# Autodesk Inventor assembly: Idler Front-Unit [B]
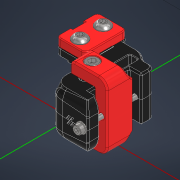
[picture p0: Inventor's stored thumbnail of the model, 180x180]
Saved by Autodesk Inventor 2022.2 (Build 262287010, 287A)
## iProperties
Created: 2022-03-14
Part Number: Idler Front-Unit [B]
Document SubType Name: Assembly
Designer: sleib
Author: sleib
## Documents named in this file (10)
- C:\Users\sleib\Projekte\Voron-2\CAD\Inventor\Idler Front-Unit [B].iam
- C:\Users\sleib\Projekte\Voron-2\CAD\Inventor\Idler Front Top [B].ipt
- C:\Users\sleib\Projekte\Voron-2\CAD\Inventor\Idler Front Bottom [B].ipt
- C:\Users\sleib\Projekte\Voron-2\CAD\Inventor\Idler Front Tensioner-Unit [B].iam
- C:\Users\sleib\Projekte\Voron-2\CAD\Inventor\M3x40 SHCS.ipt
- C:\Users\sleib\Projekte\Voron-2\CAD\Inventor\M5 Spacer (1mm).ipt
- C:\Users\sleib\Projekte\Voron-2\CAD\Inventor\Bearing F695-ZZ.ipt
- C:\Users\sleib\Projekte\Voron-2\CAD\Inventor\Z Belt-Clamp Upper.ipt
- C:\Users\sleib\Projekte\Voron-2\CAD\Inventor\M5x16 BHCS.ipt
- C:\Users\sleib\Projekte\Voron-2\CAD\Inventor\M3 Washer.ipt
## Components (12 placed, 9 different names)
1. Idler Front Top [B]:1 — Passend:1, Passend:3, Passend:5, Passend:6, Fluchtend:1, Winkel:1, Passend:8, Passend:11, Passend:19, Passend:22, Passend:25, Passend:26
2. Idler Front Bottom [B]:1 — Passend:5, Passend:6, Fluchtend:1, Passend:30, Passend:32
3. Idler Front Tensioner-Unit [B]:1 [sub-assembly] — Winkel:1, Passend:9, Passend:11, Passend:12, Passend:13, Passend:14, Passend:15
4. M3x40 SHCS:1 — Passend:8, Passend:9, Passend:29, Passend:31
5. M5 Spacer (1mm):1 — Passend:12, Passend:18, Passend:19
6. M5 Spacer (1mm):2 — Passend:15, Passend:16
7. Bearing F695-ZZ:1 — Passend:13, Passend:17, Passend:18
8. Bearing F695-ZZ:2 — Passend:14, Passend:16, Passend:17
9. Z Belt-Clamp Upper:1 — Passend:22, Passend:23, Passend:24, Passend:27, Passend:28
10. M5x16 BHCS:1 — Passend:23, Passend:25, Passend:27
11. M5x16 BHCS:2 — Passend:24, Passend:26, Passend:28
12. M3 Washer:1 — Passend:29, Passend:30, Passend:31
## Relationships (28: Mate 26, Flush 1, Angle 1)
- Passend:1 [Mate]: Idler Front Top [B]:1
- Passend:3 [Mate]: Idler Front Top [B]:1
- Passend:5 [Mate]: Idler Front Top [B]:1 ↔ Idler Front Bottom [B]:1
- Passend:6 [Mate]: Idler Front Top [B]:1 ↔ Idler Front Bottom [B]:1
- Fluchtend:1 [Flush]: Idler Front Top [B]:1 ↔ Idler Front Bottom [B]:1
- Winkel:1 [Angle] (0 deg): Idler Front Top [B]:1 ↔ Idler Front Tensioner-Unit [B]:1
- Passend:8 [Mate]: Idler Front Top [B]:1 ↔ M3x40 SHCS:1
- Passend:9 [Mate]: Idler Front Tensioner-Unit [B]:1 ↔ M3x40 SHCS:1
- Passend:11 [Mate] (5 mm): Idler Front Top [B]:1 ↔ Idler Front Tensioner-Unit [B]:1
- Passend:12 [Mate]: Idler Front Tensioner-Unit [B]:1 ↔ M5 Spacer (1mm):1
- Passend:13 [Mate]: Idler Front Tensioner-Unit [B]:1 ↔ Bearing F695-ZZ:1
- Passend:14 [Mate]: Idler Front Tensioner-Unit [B]:1 ↔ Bearing F695-ZZ:2
- Passend:15 [Mate]: Idler Front Tensioner-Unit [B]:1 ↔ M5 Spacer (1mm):2
- Passend:16 [Mate]: M5 Spacer (1mm):2 ↔ Bearing F695-ZZ:2
- Passend:17 [Mate]: Bearing F695-ZZ:1 ↔ Bearing F695-ZZ:2
- Passend:18 [Mate]: M5 Spacer (1mm):1 ↔ Bearing F695-ZZ:1
- Passend:19 [Mate]: Idler Front Top [B]:1 ↔ M5 Spacer (1mm):1
- Passend:22 [Mate]: Idler Front Top [B]:1 ↔ Z Belt-Clamp Upper:1
- Passend:23 [Mate]: Z Belt-Clamp Upper:1 ↔ M5x16 BHCS:1
- Passend:24 [Mate]: Z Belt-Clamp Upper:1 ↔ M5x16 BHCS:2
- Passend:25 [Mate]: Idler Front Top [B]:1 ↔ M5x16 BHCS:1
- Passend:26 [Mate]: Idler Front Top [B]:1 ↔ M5x16 BHCS:2
- Passend:27 [Mate]: Z Belt-Clamp Upper:1 ↔ M5x16 BHCS:1
- Passend:28 [Mate]: Z Belt-Clamp Upper:1 ↔ M5x16 BHCS:2
- Passend:29 [Mate]: M3x40 SHCS:1 ↔ M3 Washer:1
- Passend:30 [Mate]: Idler Front Bottom [B]:1 ↔ M3 Washer:1
- Passend:31 [Mate]: M3x40 SHCS:1 ↔ M3 Washer:1
- Passend:32 [Mate]: Idler Front Bottom [B]:1
